# Autodesk Inventor assembly: FingerGeneric
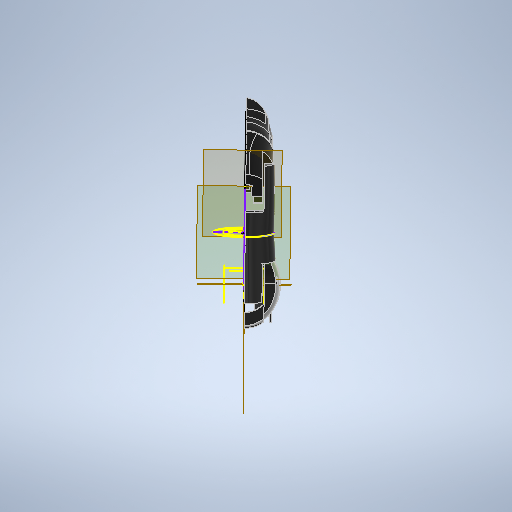
[picture p0: Inventor's stored thumbnail of the model, 512x512]
Saved by Autodesk Inventor 2025.1 (Build 291241000, 241)
## iProperties
Created: 2024-09-11
Part Number: FingerGeneric
Document SubType Name: Assembly
Designer: Alexander
Author: Alexander
## Documents named in this file (11)
- D:\Repositorios_Politecnica\Handi-EPN\CAD\Sim Models\FingerGeneric.iam
- D:\Repositorios_Politecnica\Handi-EPN\CAD\Right Finger\DP - D Tip.ipt
- D:\Repositorios_Politecnica\Handi-EPN\CAD\Right Finger\DP - D FSR Actuator.ipt
- D:\Repositorios_Politecnica\Handi-EPN\CAD\Right Finger\DP - D Lock.ipt
- D:\Repositorios_Politecnica\Handi-EPN\CAD\Right Finger\DP - D Main.ipt
- D:\Repositorios_Politecnica\Handi-EPN\CAD\Right Finger\DP - P Main R.ipt
- D:\Repositorios_Politecnica\Handi-EPN\CAD\Right Finger\PP - P MainD2 R.ipt
- D:\Repositorios_Politecnica\Handi-EPN\CAD\Right Finger\PP - P PivotD2 R.ipt
- D:\Repositorios_Politecnica\Handi-EPN\CAD\Right Finger\IP - D R.ipt
- D:\Repositorios_Politecnica\Handi-EPN\CAD\Right Finger\IP - P Main R.ipt
- D:\Repositorios_Politecnica\Handi-EPN\CAD\Right Finger\PP - D R.ipt
## Components (10 placed, 10 different names)
1. DP - D Tip:1 — Mate:3, Mate:4, Flush:1
2. DP - D FSR Actuator:1 — Mate:1, Mate:2, Mate:4
3. DP - D Lock:1 — Mate:5, Flush:2, Flush:3, Angle:1, Mate:20, Mate:21
4. DP - D Main:1 — Mate:1, Mate:2, Mate:3, Flush:1, Mate:5, Flush:2, Flush:3
5. DP - P Main R:1 — Angle:1, Rotational:1, Mate:20, Mate:21
6. PP - P MainD2 R:1 — Flush:6, Mate:17, Mate:18, Rotational:3, Symmetry:1
7. PP - P PivotD2 R:1 — Rotational:3, Symmetry:1
8. IP - D R:1 — Mate:11, Mate:12, Mate:13, Rotational:1
9. IP - P Main R:1 — Mate:11, Mate:12, Mate:13, Mate:16, Rotational:2
10. PP - D R:1 — Mate:16, Flush:6, Mate:17, Mate:18, Rotational:2
## Relationships (22: Mate 13, Flush 4, RevoluteJoint 3, Angle 1, Symmetry 1)
- Mate:1: DP - D FSR Actuator:1 ↔ DP - D Main:1
- Mate:2: DP - D FSR Actuator:1 ↔ DP - D Main:1
- Mate:3: DP - D Tip:1 ↔ DP - D Main:1
- Mate:4: DP - D Tip:1 ↔ DP - D FSR Actuator:1
- Flush:1: DP - D Tip:1 ↔ DP - D Main:1
- Mate:5: DP - D Lock:1 ↔ DP - D Main:1
- Flush:2: DP - D Lock:1 ↔ DP - D Main:1
- Flush:3: DP - D Lock:1 ↔ DP - D Main:1
- Angle:1 (180 deg): DP - D Lock:1 ↔ DP - P Main R:1
- Mate:11: IP - D R:1 ↔ IP - P Main R:1
- Mate:12: IP - D R:1 ↔ IP - P Main R:1
- Mate:13: IP - D R:1 ↔ IP - P Main R:1
- Mate:16: IP - P Main R:1 ↔ PP - D R:1
- Flush:6: PP - P MainD2 R:1 ↔ PP - D R:1
- Mate:17: PP - P MainD2 R:1 ↔ PP - D R:1
- Mate:18: PP - P MainD2 R:1 ↔ PP - D R:1
- Rotational:1 [RevoluteJoint]: DP - P Main R:1 ↔ IP - D R:1
- Mate:20: DP - D Lock:1 ↔ DP - P Main R:1
- Mate:21: DP - D Lock:1 ↔ DP - P Main R:1
- Rotational:2 [RevoluteJoint]: IP - P Main R:1 ↔ PP - D R:1
- Rotational:3 [RevoluteJoint]: PP - P MainD2 R:1 ↔ PP - P PivotD2 R:1
- Symmetry:1: PP - P MainD2 R:1 ↔ PP - P PivotD2 R:1
